# Autodesk Inventor assembly: AluminumChannelRight
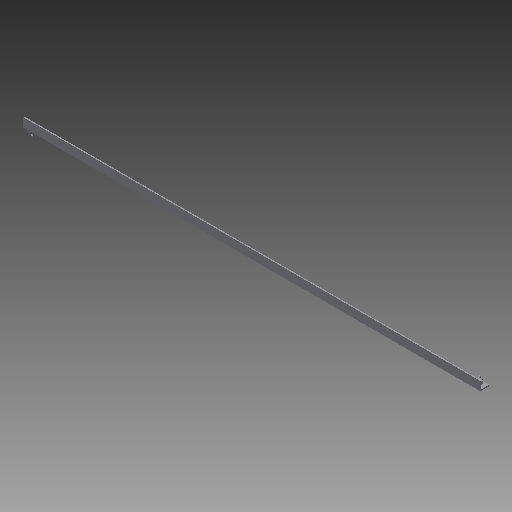
[picture p0: Inventor's stored thumbnail of the model, 512x512]
Saved by Autodesk Inventor 2019.4 (Build 234330000, 330)
## iProperties
Created: 2019-01-24
Part Number: AluminumChannelRight
Document SubType Name: Assembly
Designer: josh
Mass: 91.141 g
Surface Area: 782.59 cm^2
Volume: 91.141 cm^3
Density: 1 g/cm^3
Author: josh
## Documents named in this file (4)
- D:\FIRST FRC\Synthesis Robots\Epsilon\Chasis\AluminumChannelRight.iam
- D:\FIRST FRC\Synthesis Robots\Epsilon\Chasis\AluminumLchannel.ipt
- D:\FIRST FRC\Synthesis Robots\Epsilon\Swerve drive parts\10-24 Hex Washer Rolling x 3-4_93882A213.ipt
- D:\FIRST FRC\Synthesis Robots\Epsilon\Swerve drive parts\10-32 Nylock Nut 1_90631A411.ipt
## Components (5 placed, 3 different names)
1. AluminumLchannel:1 — Mate:1, Mate:2, Mate:3, Tangent:1, Tangent:2, Mate:4, Tangent:3, Tangent:4, Mate:7, Mate:8
2. 10-24 Hex Washer Rolling x 3-4_93882A213:1 — Mate:3, Tangent:1, Tangent:2, Mate:6
3. 10-24 Hex Washer Rolling x 3-4_93882A213:2 — Mate:4, Tangent:3, Tangent:4, Mate:5
4. 10-32 Nylock Nut 1_90631A411:1 — Mate:6, Mate:7
5. 10-32 Nylock Nut 1_90631A411:2 — Mate:5, Mate:8
## Relationships (12: Mate 8, Tangent 4)
- Mate:1: AluminumLchannel:1
- Mate:2: AluminumLchannel:1
- Mate:3: AluminumLchannel:1 ↔ 10-24 Hex Washer Rolling x 3-4_93882A213:1
- Tangent:1 (4.7625 mm): AluminumLchannel:1 ↔ 10-24 Hex Washer Rolling x 3-4_93882A213:1
- Tangent:2 (4.7625 mm): AluminumLchannel:1 ↔ 10-24 Hex Washer Rolling x 3-4_93882A213:1
- Mate:4: AluminumLchannel:1 ↔ 10-24 Hex Washer Rolling x 3-4_93882A213:2
- Tangent:3 (4.7625 mm): AluminumLchannel:1 ↔ 10-24 Hex Washer Rolling x 3-4_93882A213:2
- Tangent:4 (4.7625 mm): AluminumLchannel:1 ↔ 10-24 Hex Washer Rolling x 3-4_93882A213:2
- Mate:5: 10-24 Hex Washer Rolling x 3-4_93882A213:2 ↔ 10-32 Nylock Nut 1_90631A411:2
- Mate:6: 10-24 Hex Washer Rolling x 3-4_93882A213:1 ↔ 10-32 Nylock Nut 1_90631A411:1
- Mate:7 (3.175 mm): AluminumLchannel:1 ↔ 10-32 Nylock Nut 1_90631A411:1
- Mate:8 (3.175 mm): AluminumLchannel:1 ↔ 10-32 Nylock Nut 1_90631A411:2
